# Autodesk Inventor assembly: Assembly1
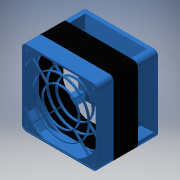
[picture p0: Inventor's stored thumbnail of the model, 180x180]
Saved by Autodesk Inventor 2016 (Build 200138000, 138)
## iProperties
Created: 2015-10-01
Part Number: Assembly1
Document SubType Name: Assembly
Designer: xdlea
Author: xdlea
## Documents named in this file (5)
- D:\Library\Documents\7-Git\3D_Printed_AirFilter\Filter Assembly.iam
- D:\Library\Documents\7-Git\3D_Printed_AirFilter\120mm Fan.ipt
- D:\Library\Documents\7-Git\3D_Printed_AirFilter\Exhaust v3.ipt
- D:\Library\Documents\7-Git\3D_Printed_AirFilter\Filter Frame.ipt
- D:\Library\Documents\7-Git\3D_Printed_AirFilter\Intake v2.ipt
## Components (4 placed, 4 different names)
1. 120mm Fan:1 — Mate:1, Mate:2, Mate:3, Mate:4, Mate:5, Mate:6, Mate:7, Mate:8, Mate:9
2. Exhaust v3:1 — Mate:4, Mate:5, Mate:6
3. Filter Frame:1 — Mate:7, Mate:8, Mate:9, Mate:10, Mate:11, Angle:1
4. Intake v2:1 — Mate:10, Mate:11, Angle:1
## Relationships (12: Mate 11, Angle 1)
- Mate:1: 120mm Fan:1
- Mate:2: 120mm Fan:1
- Mate:3: 120mm Fan:1
- Mate:4: 120mm Fan:1 ↔ Exhaust v3:1
- Mate:5: 120mm Fan:1 ↔ Exhaust v3:1
- Mate:6: 120mm Fan:1 ↔ Exhaust v3:1
- Mate:7: 120mm Fan:1 ↔ Filter Frame:1
- Mate:8: 120mm Fan:1 ↔ Filter Frame:1
- Mate:9: 120mm Fan:1 ↔ Filter Frame:1
- Mate:10: Filter Frame:1 ↔ Intake v2:1
- Mate:11: Filter Frame:1 ↔ Intake v2:1
- Angle:1 (0 deg): Filter Frame:1 ↔ Intake v2:1
